# Autodesk Inventor assembly: UpperBody
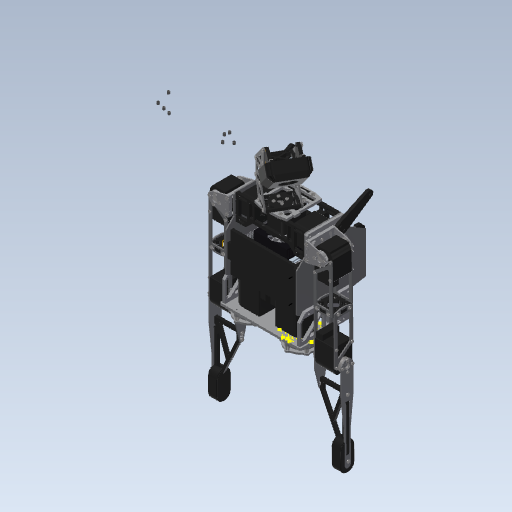
[picture p0: Inventor's stored thumbnail of the model, 512x512]
Saved by Autodesk Inventor 2020.4 (Build 244396000, 396)
## iProperties
Created: 2016-05-03
Part Number: UpperBody
Document SubType Name: Assembly
Designer: hiroaki
Mass: 2450.59 g
Surface Area: 8110.23 cm^2
Volume: 1381.3 cm^3
Density: 1.77412 g/cm^3
Author: hiroaki
## Documents named in this file (7)
- C:\Users\Masato\Documents\Inventor\CIT Brains_Inventor\OpenPlatform_ver3_0 - ve4_1 branch\UpperBody\UpperBody.iam
- C:\Users\Masato\Documents\Inventor\CIT Brains_Inventor\OpenPlatform_ver3_0 - ve4_1 branch\UpperBody\Trunk\Trunk.iam
- C:\Users\Masato\Documents\Inventor\CIT Brains_Inventor\OpenPlatform_ver3_0 - ve4_1 branch\UpperBody\Arm\ForeArm.iam
- C:\Users\Masato\Documents\Inventor\CIT Brains_Inventor\OpenPlatform_ver3_0 - ve4_1 branch\UpperBody\Arm\Shoulder.iam
- C:\Users\Masato\Documents\Inventor\CIT Brains_Inventor\OpenPlatform_ver3_0 - ve4_1 branch\UpperBody\Arm\UpperArm.iam
- C:\Users\Masato\Documents\Inventor\CIT Brains_Inventor\OpenPlatform_ver3_0 - ve4_1 branch\UpperBody\Arm\UpperArm_MIR.iam
- C:\Users\Masato\Documents\Inventor\CIT Brains_Inventor\OpenPlatform_ver3_0 - ve4_1 branch\UpperBody\Head\Head_.iam
## Components (8 placed, 6 different names)
1. Trunk:1 [sub-assembly] — 挿入:22, 挿入:23, 角度:24, 挿入:104
2. ForeArm:1 [sub-assembly] — 挿入:102, 挿入:103, 角度:27
3. Shoulder:1 [sub-assembly] — 挿入:22, 角度:23, 角度:24, 挿入:100, 挿入:101
4. Shoulder:2 [sub-assembly] — 挿入:23, 角度:23, 挿入:96, 挿入:97, 角度:25
5. UpperArm_MIR:1 [sub-assembly] — 挿入:96, 挿入:97, 挿入:98, 挿入:99, 角度:25, 角度:26
6. ForeArm:2 [sub-assembly] — 挿入:98, 挿入:99, 角度:26
7. UpperArm:1 [sub-assembly] — 挿入:100, 挿入:101, 挿入:102, 挿入:103, 角度:27
8. Head_:1 [sub-assembly] — 挿入:104
## Relationships (16: Insert 11, Angle 5)
- 挿入:22 [Insert]: Trunk:1 ↔ Shoulder:1
- 挿入:23 [Insert]: Trunk:1 ↔ Shoulder:2
- 角度:23 [Angle] (0 deg): Shoulder:1 ↔ Shoulder:2
- 角度:24 [Angle] (0 deg): Trunk:1 ↔ Shoulder:1
- 挿入:96 [Insert]: Shoulder:2 ↔ UpperArm_MIR:1
- 挿入:97 [Insert]: Shoulder:2 ↔ UpperArm_MIR:1
- 挿入:98 [Insert]: UpperArm_MIR:1 ↔ ForeArm:2
- 挿入:99 [Insert]: UpperArm_MIR:1 ↔ ForeArm:2
- 挿入:100 [Insert]: Shoulder:1 ↔ UpperArm:1
- 挿入:101 [Insert]: Shoulder:1 ↔ UpperArm:1
- 挿入:102 [Insert]: ForeArm:1 ↔ UpperArm:1
- 挿入:103 [Insert]: ForeArm:1 ↔ UpperArm:1
- 挿入:104 [Insert]: Trunk:1 ↔ Head_:1
- 角度:25 [Angle] (0 deg): Shoulder:2 ↔ UpperArm_MIR:1
- 角度:26 [Angle] (0 deg): UpperArm_MIR:1 ↔ ForeArm:2
- 角度:27 [Angle] (0 deg): ForeArm:1 ↔ UpperArm:1
